# Autodesk Inventor assembly: Assembly1
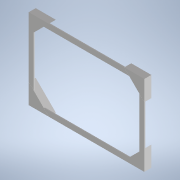
[picture p0: Inventor's stored thumbnail of the model, 180x180]
Saved by Autodesk Inventor 2020 (Build 240168000, 168)
## iProperties
Created: 2020-07-03
Part Number: Assembly1
Document SubType Name: Assembly
Designer: user
Author: user
## Documents named in this file (4)
- C:\Users\user\Documents\Github\3D_Designs\BonsaiFeet\Assembly1.iam
- C:\Users\user\Documents\Github\3D_Designs\BonsaiFeet\BonsaiFeet.ipt
- C:\Users\user\Documents\Github\3D_Designs\MagicTokenHolder\models\Bridge_Width.ipt
- C:\Users\user\Documents\Github\3D_Designs\BonsaiFeet\Bridge_width_small.ipt
## Components (8 placed, 3 different names)
1. BonsaiFeet:1 — Mate:1, Flush:1, Flush:3, Flush:4, Mate:6, Flush:12, Flush:13, Flush:16, Flush:17
2. BonsaiFeet:2 — Mate:4, Flush:8, Flush:9, Mate:7, Flush:14
3. BonsaiFeet:3 — Mate:3, Flush:6, Flush:7, Flush:15
4. BonsaiFeet:4 — Mate:2, Flush:2, Flush:3, Flush:5, Mate:5, Flush:10, Flush:11
5. Bridge_Width:1 — Mate:1, Flush:1, Mate:2, Flush:2, Flush:4, Flush:5, Flush:16, Flush:17
6. Bridge_Width:2 — Mate:3, Flush:6, Flush:7, Mate:4, Flush:8, Flush:9
7. Bridge_width_small:1 — Mate:5, Flush:10, Flush:11, Flush:15
8. Bridge_width_small:2 — Mate:6, Flush:12, Flush:13, Mate:7, Flush:14
## Relationships (24: Flush 17, Mate 7)
- Mate:1: BonsaiFeet:1 ↔ Bridge_Width:1
- Flush:1: BonsaiFeet:1 ↔ Bridge_Width:1
- Mate:2: BonsaiFeet:4 ↔ Bridge_Width:1
- Flush:2: BonsaiFeet:4 ↔ Bridge_Width:1
- Flush:3: BonsaiFeet:1 ↔ BonsaiFeet:4
- Flush:4: BonsaiFeet:1 ↔ Bridge_Width:1
- Flush:5: BonsaiFeet:4 ↔ Bridge_Width:1
- Mate:3: BonsaiFeet:3 ↔ Bridge_Width:2
- Flush:6: BonsaiFeet:3 ↔ Bridge_Width:2
- Flush:7: BonsaiFeet:3 ↔ Bridge_Width:2
- Mate:4: BonsaiFeet:2 ↔ Bridge_Width:2
- Flush:8: BonsaiFeet:2 ↔ Bridge_Width:2
- Flush:9: BonsaiFeet:2 ↔ Bridge_Width:2
- Mate:5: BonsaiFeet:4 ↔ Bridge_width_small:1
- Flush:10: BonsaiFeet:4 ↔ Bridge_width_small:1
- Flush:11: BonsaiFeet:4 ↔ Bridge_width_small:1
- Mate:6: BonsaiFeet:1 ↔ Bridge_width_small:2
- Flush:12: BonsaiFeet:1 ↔ Bridge_width_small:2
- Flush:13: BonsaiFeet:1 ↔ Bridge_width_small:2
- Mate:7: BonsaiFeet:2 ↔ Bridge_width_small:2
- Flush:14: BonsaiFeet:2 ↔ Bridge_width_small:2
- Flush:15: BonsaiFeet:3 ↔ Bridge_width_small:1
- Flush:16: BonsaiFeet:1 ↔ Bridge_Width:1
- Flush:17: BonsaiFeet:1 ↔ Bridge_Width:1
